# Autodesk Inventor assembly: e3d_v6
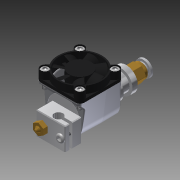
[picture p0: Inventor's stored thumbnail of the model, 180x180]
Saved by Autodesk Inventor 2013 (Build 170138000, 138)
## iProperties
Created: 2015-02-20
Part Number: e3d_v6
Document SubType Name: Assembly
Designer: Noa Izumi
Author: Noa Izumi
## Documents named in this file (10)
- C:\reprap\TinyBoy_v3_20150220\e3d_v6.iam
- C:\reprap\TinyBoy_v3_20150220\e3d_v6_heat_sink.ipt
- C:\reprap\TinyBoy_v3_20150220\e3d_v6_heat_block.ipt
- C:\reprap\TinyBoy_v3_20150220\e3d_v6_heat_break.ipt
- C:\reprap\TinyBoy_v3_20150220\e3d_v6_nozzle.ipt
- C:\reprap\TinyBoy_v3_20150220\screw_M3_10_hex.ipt
- C:\reprap\TinyBoy_v3_20150220\screw_M3_6_hex.ipt
- C:\reprap\TinyBoy_v3_20150220\e3d_v6_fan_duct.ipt
- C:\reprap\TinyBoy_v3_20150220\fan_3007.iam
- C:\reprap\TinyBoy_v3_20150220\pc4_m10.ipt
## Components (13 placed, 9 different names)
1. e3d_v6_heat_sink:1 — 插入:1, 插入:6, 插入:13
2. e3d_v6_heat_block:1 — 插入:2, 角度:1, 插入:4, 插入:5, 角度:2
3. e3d_v6_heat_break:1 — 插入:1, 插入:3
4. e3d_v6_nozzle:1 — 插入:2, 角度:1, 插入:3
5. screw_M3_10_hex:1 — 插入:4
6. screw_M3_6_hex:1 — 插入:5
7. e3d_v6_fan_duct:1 — 插入:6, 角度:2, 插入:7, 插入:8
8. fan_3007:1 [sub-assembly] — 插入:7, 插入:8, 插入:9, 插入:10, 插入:11, 插入:12
9. screw_M3_10_hex:2 — 插入:9
10. screw_M3_10_hex:3 — 插入:10
11. screw_M3_10_hex:4 — 插入:11
12. screw_M3_10_hex:5 — 插入:12
13. pc4_m10:1 — 插入:13
## Relationships (15: Insert 13, Angle 2)
- 插入:1 [Insert] (-0.1 mm): e3d_v6_heat_sink:1 ↔ e3d_v6_heat_break:1
- 插入:2 [Insert]: e3d_v6_heat_block:1 ↔ e3d_v6_nozzle:1
- 角度:1 [Angle] (0 deg): e3d_v6_heat_block:1 ↔ e3d_v6_nozzle:1
- 插入:3 [Insert]: e3d_v6_heat_break:1 ↔ e3d_v6_nozzle:1
- 插入:4 [Insert]: e3d_v6_heat_block:1 ↔ screw_M3_10_hex:1
- 插入:5 [Insert]: e3d_v6_heat_block:1 ↔ screw_M3_6_hex:1
- 插入:6 [Insert]: e3d_v6_heat_sink:1 ↔ e3d_v6_fan_duct:1
- 角度:2 [Angle] (0 deg): e3d_v6_heat_block:1 ↔ e3d_v6_fan_duct:1
- 插入:7 [Insert]: e3d_v6_fan_duct:1 ↔ fan_3007:1
- 插入:8 [Insert]: e3d_v6_fan_duct:1 ↔ fan_3007:1
- 插入:9 [Insert]: fan_3007:1 ↔ screw_M3_10_hex:2
- 插入:10 [Insert]: fan_3007:1 ↔ screw_M3_10_hex:3
- 插入:11 [Insert]: fan_3007:1 ↔ screw_M3_10_hex:4
- 插入:12 [Insert]: fan_3007:1 ↔ screw_M3_10_hex:5
- 插入:13 [Insert]: e3d_v6_heat_sink:1 ↔ pc4_m10:1
